# Autodesk Inventor assembly: s5 mini basr r1
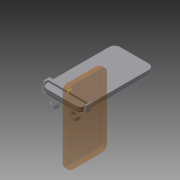
[picture p0: Inventor's stored thumbnail of the model, 180x180]
Saved by Autodesk Inventor 2017 (Build 210142000, 142)
## iProperties
Created: 2017-06-10
Part Number: s5 mini basr r1
Document SubType Name: Assembly
Designer: ari
Author: ari
## Documents named in this file (3)
- C:\Users\ari\Documents\Inventor\s5 mini\s5 mini basr r1.iam
- C:\Users\ari\Documents\Inventor\s5 mini\basic shape.ipt
- C:\Users\ari\Documents\Inventor\s5 mini\holder_bottom.ipt
## Components (2 placed, 2 different names)
1. basic shape:1 — Flush:1
2. holder_bottom:1 — Flush:1
## Relationships (1: Flush 1)
- Flush:1: basic shape:1 ↔ holder_bottom:1
